# Autodesk Inventor assembly: frameSides
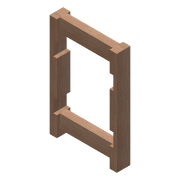
[picture p0: Inventor's stored thumbnail of the model, 180x180]
Saved by Autodesk Inventor 2018 (Build 220112000, 112)
## iProperties
Created: 2018-01-02
Part Number: frameSides
Document SubType Name: Assembly
Designer: sawaiz
Author: sawaiz
## Documents named in this file (4)
- C:\Users\sawaiz\OneDrive\personal\berlin\Move\larkspur\kitchen\frameSides.iam
- C:\Users\sawaiz\OneDrive\personal\berlin\Move\larkspur\kitchen\frameVertical.ipt
- C:\Users\sawaiz\OneDrive\personal\berlin\Move\larkspur\kitchen\frameDepth.ipt
- C:\Users\sawaiz\OneDrive\personal\berlin\Move\larkspur\kitchen\kitchen.xlsx
## Components (4 placed, 2 different names)
1. frameVertical:1 — Mate:4, Flush:1, Flush:6, Flush:8, Flush:9, Flush:10, Mate:6, Flush:12, Symmetry:2, Symmetry:3
2. frameVertical:2 — Flush:1, Mate:5, Flush:9, Flush:10, Symmetry:2, Symmetry:3
3. frameDepth:1 — Flush:4, Flush:6, Mate:5, Mate:6, Flush:11, Flush:12, Symmetry:1
4. frameDepth:2 — Mate:4, Flush:4, Flush:8, Flush:11, Symmetry:1
## Relationships (14: Flush 8, Mate 3, Symmetry 3)
- Mate:4: frameVertical:1 ↔ frameDepth:2
- Flush:1: frameVertical:1 ↔ frameVertical:2
- Flush:4: frameDepth:1 ↔ frameDepth:2
- Flush:6: frameVertical:1 ↔ frameDepth:1
- Flush:8 (50 mm): frameVertical:1 ↔ frameDepth:2
- Mate:5: frameVertical:2 ↔ frameDepth:1
- Flush:9: frameVertical:1 ↔ frameVertical:2
- Flush:10: frameVertical:1 ↔ frameVertical:2
- Mate:6: frameVertical:1 ↔ frameDepth:1
- Flush:11: frameDepth:1 ↔ frameDepth:2
- Flush:12 (25 mm): frameVertical:1 ↔ frameDepth:1
- Symmetry:1: frameDepth:1 ↔ frameDepth:2
- Symmetry:2: frameVertical:1 ↔ frameVertical:2
- Symmetry:3: frameVertical:1 ↔ frameVertical:2
## Named parameters: lumberWidth = 58 mm, lumberDepth = 108 mm, counterThickness = 38 mm, frameHeight = 820 mm, counterHeight = 858 mm, counterDepth = 635 mm, frameOverhang = 50 mm
